# Autodesk Inventor assembly: ConnectionBox
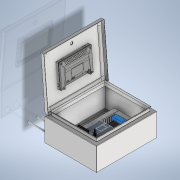
[picture p0: Inventor's stored thumbnail of the model, 180x180]
Saved by Autodesk Inventor 2022 (Build 260153000, 153)
## iProperties
Created: 2024-10-26
Part Number: ConnectionBox
Document SubType Name: Assembly
Designer: NANOmatic
Author: NANOmatic
## Documents named in this file (12)
- C:\Users\NANOmatic\Downloads\TomaszGwizdak\3D\ControlUnit.iam
- C:\Users\NANOmatic\Downloads\TomaszGwizdak\3D\TH35.ipt
- C:\Users\NANOmatic\Downloads\TomaszGwizdak\3D\HDR-60-24.ipt
- C:\Users\NANOmatic\Downloads\TomaszGwizdak\3D\PLC\6ES7214-1AG40-0XB0.iam
- C:\Users\NANOmatic\Downloads\TomaszGwizdak\3D\HMI\MT8072iP.iam
- C:\Users\NANOmatic\Downloads\TomaszGwizdak\3D\RB941-2nD.ipt
- C:\Users\NANOmatic\Downloads\TomaszGwizdak\3D\ECS2540\ECS2540.iam
- C:\Users\NANOmatic\Downloads\TomaszGwizdak\3D\CJ-ACI.ipt
- C:\Users\NANOmatic\Downloads\TomaszGwizdak\3D\F1.0256\F1.0256.iam
- C:\Users\NANOmatic\Downloads\TomaszGwizdak\3D\ECS2540\ECS2540_CPY.iam
- C:\Users\NANOmatic\Downloads\TomaszGwizdak\3D\PG11.ipt
- C:\Users\NANOmatic\Downloads\TomaszGwizdak\3D\Cable.ipt
## Components (15 placed, 11 different names)
1. TH35:1 — Zestawiające:1, Równoległe:1, Zestawiające:2, Równoległe:2, Zestawiające:4, Równoległe:3, Zestawiające:6, Kątowe:6, Zestawiające:9, Równoległe:14, Równoległe:19, Równoległe:21
2. HDR-60-24:1 — Zestawiające:1, Równoległe:1, Zestawiające:3, Zestawiające:5
3. 6ES7214-1AG40-0XB0:1 [sub-assembly] — Zestawiające:2, Równoległe:2, Zestawiające:3, Zestawiające:7
4. MT8072iP:1 [sub-assembly] — Zestawiające:10, Zestawiające:11
5. RB941-2nD:1 — Zestawiające:6, Zestawiające:7, Równoległe:14
6. ECS2540:1 [sub-assembly] — Kątowe:6, Równoległe:15, Równoległe:16, Zestawiające:12, Symetria:1
7. CJ-ACI:1 — Zestawiające:4, Równoległe:3, Zestawiające:5
8. F1.0256:1 [sub-assembly] — Zestawiające:9, Równoległe:11, Równoległe:12, Równoległe:13, Zestawiające:10, Zestawiające:11, Równoległe:15, Równoległe:16, Zestawiające:12, Zestawiające:13, Równoległe:18, Równoległe:19, Zestawiające:14, Równoległe:20, Równoległe:21, Zestawiające:16, Równoległe:22, Zestawiające:18, Zestawiające:19, Symetria:2, Zestawiające:26
9. ECS2540:2 [sub-assembly] — Zestawiające:13, Równoległe:18, Symetria:1, Zestawiające:15, Zestawiające:17, Zestawiające:23, Zestawiające:24, Symetria:2
10. ECS2540_CPY:1 [sub-assembly] — Zestawiające:14, Równoległe:20, Zestawiające:15
11. ECS2540_CPY:2 [sub-assembly] — Zestawiające:16, Równoległe:22, Zestawiające:17
12. PG11:1 — Zestawiające:18, Zestawiające:20, Zestawiające:22, Zestawiające:25, Zestawiające:26
13. PG11:2 — Zestawiające:19, Zestawiające:20, Zestawiające:21, Zestawiające:25
14. Cable:1 — Zestawiające:21, Zestawiające:24
15. Cable:2 — Zestawiające:22, Zestawiające:23
## Relationships (42: Mate 25, Flush 14, Symmetry 2, Angle 1)
- Zestawiające:1 [Mate]: TH35:1 ↔ HDR-60-24:1
- Równoległe:1 [Flush]: TH35:1 ↔ HDR-60-24:1
- Zestawiające:2 [Mate]: TH35:1 ↔ 6ES7214-1AG40-0XB0:1
- Równoległe:2 [Flush]: TH35:1 ↔ 6ES7214-1AG40-0XB0:1
- Zestawiające:3 [Mate]: HDR-60-24:1 ↔ 6ES7214-1AG40-0XB0:1
- Zestawiające:4 [Mate]: TH35:1 ↔ CJ-ACI:1
- Równoległe:3 [Flush]: TH35:1 ↔ CJ-ACI:1
- Zestawiające:5 [Mate] (10 mm): HDR-60-24:1 ↔ CJ-ACI:1
- Zestawiające:6 [Mate] (5 mm): TH35:1 ↔ RB941-2nD:1
- Zestawiające:7 [Mate]: 6ES7214-1AG40-0XB0:1 ↔ RB941-2nD:1
- Kątowe:6 [Angle] (0 deg): TH35:1 ↔ ECS2540:1
- Zestawiające:9 [Mate]: TH35:1 ↔ F1.0256:1
- Równoległe:11 [Flush]: F1.0256:1
- Równoległe:12 [Flush]: F1.0256:1
- Równoległe:13 [Flush]: F1.0256:1
- Równoległe:14 [Flush]: TH35:1 ↔ RB941-2nD:1
- Zestawiające:10 [Mate]: MT8072iP:1 ↔ F1.0256:1
- Zestawiające:11 [Mate]: MT8072iP:1 ↔ F1.0256:1
- Równoległe:15 [Flush]: ECS2540:1 ↔ F1.0256:1
- Równoległe:16 [Flush]: ECS2540:1 ↔ F1.0256:1
- Zestawiające:12 [Mate]: ECS2540:1 ↔ F1.0256:1
- Zestawiające:13 [Mate]: F1.0256:1 ↔ ECS2540:2
- Równoległe:18 [Flush]: F1.0256:1 ↔ ECS2540:2
- Równoległe:19 [Flush] (100 mm): TH35:1 ↔ F1.0256:1
- Symetria:1 [Symmetry]: ECS2540:1 ↔ ECS2540:2
- Zestawiające:14 [Mate]: F1.0256:1 ↔ ECS2540_CPY:1
- Równoległe:20 [Flush]: F1.0256:1 ↔ ECS2540_CPY:1
- Zestawiające:15 [Mate]: ECS2540:2 ↔ ECS2540_CPY:1
- Równoległe:21 [Flush]: TH35:1 ↔ F1.0256:1
- Zestawiające:16 [Mate]: F1.0256:1 ↔ ECS2540_CPY:2
- Równoległe:22 [Flush]: F1.0256:1 ↔ ECS2540_CPY:2
- Zestawiające:17 [Mate]: ECS2540:2 ↔ ECS2540_CPY:2
- Zestawiające:18 [Mate]: F1.0256:1 ↔ PG11:1
- Zestawiające:19 [Mate]: F1.0256:1 ↔ PG11:2
- Zestawiające:20 [Mate]: PG11:1 ↔ PG11:2
- Zestawiające:21 [Mate]: PG11:2 ↔ Cable:1
- Zestawiające:22 [Mate]: PG11:1 ↔ Cable:2
- Zestawiające:23 [Mate]: ECS2540:2 ↔ Cable:2
- Zestawiające:24 [Mate]: ECS2540:2 ↔ Cable:1
- Symetria:2 [Symmetry]: F1.0256:1 ↔ ECS2540:2
- Zestawiające:25 [Mate] (50 mm): PG11:1 ↔ PG11:2
- Zestawiające:26 [Mate] (-30 mm): F1.0256:1 ↔ PG11:1
